# Autodesk Inventor assembly: Assembly1
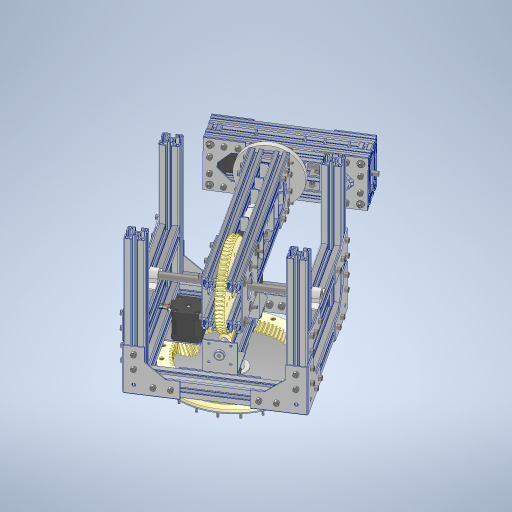
[picture p0: Inventor's stored thumbnail of the model, 512x512]
Saved by Autodesk Inventor 2024 (Build 280153000, 153)
## iProperties
Created: 2025-12-08
Part Number: Assembly1
Document SubType Name: Assembly
Designer: schar
Author: schar
## Documents named in this file (47)
- C:\Users\schar\Desktop\projectBlueprint\AMSTS\hardware\Assembly1.iam
- C:\Users\schar\Desktop\projectBlueprint\AMSTS\hardware\3030_200.ipt
- C:\Users\schar\Desktop\projectBlueprint\AMSTS\hardware\Connect2x3030_m6.ipt
- C:\Users\schar\Desktop\projectBlueprint\AMSTS\hardware\3030_tnut_m6.ipt
- C:\Users\schar\Documents\Inventor\Content Center Files\R2024\en-US\AS 1420\AS 1420 - 1973 - M5 x 10.ipt
- C:\Users\schar\Desktop\projectBlueprint\AMSTS\hardware\3030_260.ipt
- C:\Users\schar\Desktop\projectBlueprint\AMSTS\hardware\3030_connector_assembled.iam
- C:\Users\schar\Desktop\projectBlueprint\AMSTS\hardware\3030_connector_assembled_MIR.iam
- C:\Users\schar\Desktop\projectBlueprint\AMSTS\hardware\3030_connector_assembled_MIR1.iam
- C:\Users\schar\Desktop\projectBlueprint\AMSTS\hardware\3030_connector_assembled_MIR_MIR.iam
- C:\Users\schar\Desktop\projectBlueprint\AMSTS\hardware\3030_T_connector_assembled.iam
- C:\Users\schar\Desktop\projectBlueprint\AMSTS\hardware\3030_T_connector_assembled_MIR1.iam
- C:\Users\schar\Desktop\projectBlueprint\AMSTS\hardware\wormgear_pol_base.iam
- C:\Users\schar\Desktop\projectBlueprint\AMSTS\hardware\base_axis_static_12mm.ipt
- C:\Users\schar\Desktop\projectBlueprint\AMSTS\hardware\base_axis_12mm.ipt
- C:\Users\schar\Desktop\projectBlueprint\AMSTS\hardware\NEMA17-3030-m6-holder.ipt
- C:\Users\schar\Desktop\projectBlueprint\AMSTS\hardware\3030_tnut_m6_main.ipt
- C:\Users\schar\Desktop\projectBlueprint\AMSTS\hardware\basis-bearing-3030-m6-holder.ipt
- C:\Users\schar\Desktop\projectBlueprint\AMSTS\hardware\wormgear_axis_6mm.ipt
- C:\Users\schar\Desktop\projectBlueprint\AMSTS\hardware\wormgear_worm_axes_holder.ipt
- C:\Users\schar\Desktop\projectBlueprint\AMSTS\hardware\bearing_shaft_base_mount.ipt
- C:\Users\schar\Desktop\projectBlueprint\AMSTS\hardware\az_rot_plate.iam
- C:\Users\schar\Desktop\projectBlueprint\AMSTS\hardware\the_part_that_holds_everything_together.ipt
- C:\Users\schar\Desktop\projectBlueprint\AMSTS\hardware\6901.iam
- C:\Users\schar\Desktop\projectBlueprint\AMSTS\hardware\2020_400.ipt
- C:\Users\schar\Desktop\projectBlueprint\AMSTS\hardware\mount_plate_4x2020.ipt
- C:\Users\schar\Documents\Inventor\Content Center Files\R2024\en-US\DIN 9021\DIN 9021 - 5,3.ipt
- C:\Users\schar\Desktop\projectBlueprint\AMSTS\hardware\m5x70.ipt
- C:\Users\schar\Desktop\projectBlueprint\AMSTS\hardware\3030_tnut_m6_MIR3.ipt
- C:\Users\schar\Documents\Inventor\Content Center Files\R2024\en-US\ISO 4762(1)\DIN EN ISO 4762 - M6 x 10.ipt
- C:\Users\schar\Desktop\projectBlueprint\AMSTS\hardware\3030_L-Bracket_asm.ipt.iam
- C:\Users\schar\Desktop\projectBlueprint\AMSTS\hardware\4x2020_in.iam
- C:\Users\schar\Desktop\projectBlueprint\AMSTS\hardware\2020_4x2020_hz.ipt
- C:\Users\schar\Desktop\projectBlueprint\AMSTS\hardware\2020_4x2020_ve.ipt
- C:\Users\schar\Desktop\projectBlueprint\AMSTS\hardware\17HE19-2004S.ipt
- C:\Users\schar\Desktop\projectBlueprint\AMSTS\hardware\az_rot_mot_asm.ipt.iam
- C:\Users\schar\Desktop\projectBlueprint\AMSTS\hardware\azimuth_gear_in.ipt
- C:\Users\schar\Documents\Inventor\Content Center Files\R2024\en-US\DIN 913\DIN 913 - M5 x 5.ipt
- C:\Users\schar\Desktop\projectBlueprint\AMSTS\hardware\Connect_u2020_asm.iam
- C:\Users\schar\Desktop\projectBlueprint\AMSTS\hardware\m4x70_example.ipt
- C:\Users\schar\Documents\Inventor\Content Center Files\R2024\en-US\DIN 9021\DIN 9021 - 4,3.ipt
- C:\Users\schar\Desktop\projectBlueprint\AMSTS\hardware\ax4_holder_asm.iam
- C:\Users\schar\Desktop\projectBlueprint\AMSTS\hardware\4ax_plate_joint_asm.iam
- C:\Users\schar\Desktop\projectBlueprint\AMSTS\hardware\ax4.iam
- C:\Users\schar\Desktop\projectBlueprint\AMSTS\hardware\13to6_bearing.ipt
- 3030_L-Bracket_asm.ipt
- az_rot_mot_asm.ipt
## Components (125 placed, 44 different names)
1. 3030_tnut_m6_main:17 — Rotational:21
2. 3030_tnut_m6_main:18 — Rotational:22
3. bearing_shaft_base_mount:1 — Mate:102, Flush:37, Flush:38, Rotational:21, Rotational:22, Mate:103, Rotational:25
4. az_rot_plate:1 [sub-assembly] — Mate:103, Tangent:1, Rotational:23, Rotational:24, Mate:182, Insert:27, Mate:183
5. the_part_that_holds_everything_together:1 — Rotational:24, Rotational:25
6. 6901:1 [sub-assembly] — Rotational:23
7. 2020_400:1 — Mate:109, Mate:113, Mate:114, Mate:121, Mate:157, Mate:158, Mate:162, Flush:46, Flush:47, Mate:185, Mate:187, Flush:63
8. 2020_400:2 — Mate:107, Mate:117, Mate:118, Mate:122, Mate:123, Flush:56, Mate:184
9. 2020_400:3 — Mate:110, Mate:111, Mate:112, Mate:124, Flush:43, Mate:155, Mate:161, Flush:44, Flush:45
10. 2020_400:4 — Mate:108, Mate:115, Mate:116, Mate:119, Mate:120, Mate:159, Mate:160, Flush:58, Mate:186, Flush:62
11. mount_plate_4x2020:1 — Mate:119, Mate:120, Mate:121, Mate:125, Mate:150
12. mount_plate_4x2020:2 — Mate:122, Mate:123, Mate:124, Mate:154
13. 3030_L-Bracket_asm.ipt:1 [sub-assembly] — Mate:141, Flush:41, Mate:142
14. 3030_L-Bracket_asm.ipt:2 [sub-assembly] — Mate:139, Flush:40, Mate:140
15. 3030_L-Bracket_asm.ipt:3 [sub-assembly] — Mate:137, Flush:39, Mate:138
16. 3030_L-Bracket_asm.ipt:4 [sub-assembly] — Mate:143, Flush:42, Mate:144
17. 4x2020_in:1 [sub-assembly] — Flush:43, Mate:155, Mate:156, Mate:194, Mate:195, Mate:197
18. 2020_4x2020_hz:1 — Mate:159, Mate:160, Flush:62
19. 2020_4x2020_hz:2 — Mate:157, Mate:158, Flush:63
20. 2020_4x2020_ve:1 — Mate:162, Flush:46, Flush:47, Flush:59
21. 2020_4x2020_ve:2 — Mate:161, Flush:44, Flush:45, Flush:57, Mate:196
22. 17HE19-2004S:1 — Mate:165, Mate:166, Mate:167, Mate:202
23. az_rot_mot_asm.ipt:1 [sub-assembly] — Mate:181, Flush:55, Mate:182
24. 3030_tnut_m6_MIR3:1 — Mate:177, Mate:178
25. 3030_tnut_m6_MIR3:2 — Mate:179, Mate:180
26. DIN EN ISO 4762 M6 x 10:1 — Mate:174, Mate:175, Mate:177
27. DIN EN ISO 4762 M6 x 10:2 — Mate:173, Mate:176, Mate:179
28. azimuth_gear_in:1 — Rotational:31, Insert:27, Mate:183
29. DIN 913 M5 x 5:1 — Rotational:31
30. Connect_u2020_asm:1 [sub-assembly] — Flush:56, Flush:57, Mate:184, Mate:192, Mate:193
31. Connect_u2020_asm:2 [sub-assembly] — Flush:58, Flush:59, Mate:185, Mate:188, Mate:189
32. m4x70_example:1 — Mate:187, Mate:188, Mate:191
33. m4x70_example:2 — Mate:186, Mate:189, Mate:190
34. DIN 9021 4,3:1 — Mate:190, Mate:193
35. DIN 9021 4,3:2 — Mate:191, Mate:192
36. ax4_holder_asm:1 [sub-assembly] — Mate:194, Mate:195, Flush:60, Mate:198, Mate:205
37. 4ax_plate_joint_asm:1 [sub-assembly] — Mate:196, Mate:197
38. ax4:1 [sub-assembly] — Flush:60, Mate:198, Mate:205
39. 13to6_bearing:1 — Mate:200, Flush:64, Flush:65
40. 3030_200:1 — Mate:1, Mate:2, Flush:1, Flush:2, Mate:4, Flush:5, Flush:6, Mate:30, Mate:48, Mate:141, Flush:41, Mate:143, Flush:42, Flush:52, Mate:203
41. 3030_200:2 — Mate:3, Flush:3, Flush:4, Mate:6, Flush:9, Flush:10
42. Connect2x3030_m6:1 — Mate:1, Mate:2, Flush:1, Flush:2, Mate:3, Flush:3, Flush:4, Rigid:1, Rotational:5, Rotational:6, Rotational:7, Insert:11, Insert:12, Insert:14, Insert:15, Mate:19, Mate:20, Mate:21, Mate:36, Mate:37
43. Connect2x3030_m6:2 — Mate:4, Flush:5, Flush:6, Mate:5, Flush:7, Flush:8, Rotational:1, Rotational:2, Rotational:3, Rotational:4, Insert:6, Insert:7, Insert:9, Insert:10, Mate:10, Mate:11, Mate:12, Mate:32, Mate:33
44. Connect2x3030_m6:3 — Mate:8, Flush:11, Flush:12, Rotational:12, Rotational:13, Rotational:14, Rotational:15, Insert:1, Insert:2, Insert:4, Insert:5, Mate:13, Mate:14, Mate:15, Mate:40, Mate:41
45. Connect2x3030_m6:4 — Mate:6, Flush:9, Flush:10, Mate:7, Flush:13, Mate:9, Flush:14, Rotational:8, Rotational:9, Rotational:10, Rotational:11, Insert:16, Insert:17, Insert:18, Insert:20, Mate:16, Mate:17, Mate:18, Mate:23, Flush:15, Mate:25
46. 3030_200:3 — Mate:5, Flush:7, Flush:8, Mate:8, Flush:11, Flush:12, Mate:52, Angle:1, Mate:181, Flush:55
47. 3030_200:4 — Flush:13, Mate:9, Flush:14, Mate:53, Flush:23, Mate:137, Flush:39, Mate:139, Flush:40
48. 3030_connector_assembled:1 [sub-assembly] — Mate:24, Mate:25, Mate:26
49. 3030_connector_assembled:2 [sub-assembly] — Mate:22, Mate:23, Flush:15, Mate:26
50. 3030_connector_assembled_MIR:1 [sub-assembly] — Mate:27, Mate:39, Mate:40
51. 3030_connector_assembled_MIR:2 [sub-assembly] — Mate:27, Mate:38, Mate:41
52. 3030_connector_assembled_MIR1:1 [sub-assembly] — Mate:28, Mate:34, Mate:37
53. 3030_connector_assembled_MIR1:2 [sub-assembly] — Mate:28, Mate:35, Mate:36
54. 3030_connector_assembled_MIR_MIR:1 [sub-assembly] — Mate:29, Mate:30, Mate:33
55. 3030_connector_assembled_MIR_MIR:2 [sub-assembly] — Mate:29, Mate:31, Mate:32, Mate:170
56. 3030_260:1 — Mate:10, Mate:11, Mate:12, Mate:31, Mate:49, Flush:20
57. 3030_260:2 — Mate:13, Mate:14, Mate:15, Mate:38, Mate:39, Mate:42, Flush:16
58. 3030_260:3 — Mate:16, Mate:17, Mate:18, Mate:22, Mate:24, Mate:43, Flush:17, Mate:204
59. 3030_260:4 — Mate:19, Mate:20, Mate:21, Mate:34, Mate:35, Mate:50, Flush:21
60. wormgear_axis_6mm:1 — Mate:63, Mate:64, Mate:65, Flush:65, Mate:202
61. wormgear_worm_axes_holder:1 — Mate:64, Mate:65, Rotational:26
62. wormgear_pol_base:1 [sub-assembly] — Rigid:2, Mate:63, Rotational:26, Mate:107, Mate:108, Mate:109, Mate:110, Mate:111, Mate:112, Mate:113, Mate:114, Mate:115, Mate:116, Mate:117, Mate:118, Mate:156
63. base_axis_static_12mm:1 — Flush:30, Mate:57, Insert:22
64. base_axis_static_12mm:2 — Mate:58, Flush:31, Insert:21, Mate:201
65. base_axis_12mm:1 — Insert:21, Insert:22, Rigid:2
66. basis-bearing-3030-m6-holder:1 — Mate:172, Flush:54, Mate:173, Mate:174, Mate:175, Mate:176, Mate:200, Flush:64, Mate:203
67. NEMA17-3030-m6-holder:1 — Mate:59, Flush:33, Mate:165, Mate:166, Mate:167
68. 3030_T_connector_assembled:1 [sub-assembly] — Mate:43, Flush:17, Mate:56, Flush:29
69. 3030_T_connector_assembled:2 [sub-assembly] — Mate:42, Flush:16, Flush:26
70. 3030_T_connector_assembled_MIR1:1 [sub-assembly] — Mate:50, Flush:21, Mate:55, Flush:27, Flush:28
71. 3030_T_connector_assembled_MIR1:2 [sub-assembly] — Mate:49, Flush:20, Mate:54, Flush:24, Flush:25, Mate:170
72. 3030_200:5 — Mate:48, Mate:52, Flush:22, Mate:59, Flush:33, Mate:102, Flush:37, Flush:38, Mate:138, Mate:140, Mate:142, Mate:144, Flush:52, Mate:172, Flush:54, Mate:178, Mate:180
73. 3030_T_connector_assembled:4 [sub-assembly] — Mate:53, Flush:22, Flush:23
74. 3030_200:6 — Mate:55, Flush:27, Flush:28, Mate:56, Flush:29, Flush:30, Mate:57
75. 3030_200:7 — Mate:54, Flush:24, Flush:25, Flush:26, Mate:58, Flush:31, Mate:201
76. 3030_tnut_m6:1 — Rotational:12
77. 3030_tnut_m6:2 — Rotational:11
78. 3030_tnut_m6:3 — Rigid:1
79. 3030_tnut_m6:4 — Rotational:1
80. 3030_tnut_m6:5 — Rotational:13
81. 3030_tnut_m6:6 — Rotational:10
82. 3030_tnut_m6:7 — Rotational:5
83. 3030_tnut_m6:8 — Rotational:2
84. 3030_tnut_m6:9 — Rotational:15
85. 3030_tnut_m6:10 — Rotational:8
86. 3030_tnut_m6:11 — Rotational:6
87. 3030_tnut_m6:12 — Rotational:4
88. 3030_tnut_m6:13 — Rotational:14
89. 3030_tnut_m6:14 — Rotational:9
90. 3030_tnut_m6:15 — Rotational:7
91. 3030_tnut_m6:16 — Rotational:3
92. AS 1420 - Metric M5 x 10:1 — Insert:1
93. AS 1420 - Metric M5 x 10:2 — Insert:2
94. AS 1420 - Metric M5 x 10:4 — Insert:4
95. AS 1420 - Metric M5 x 10:5 — Insert:5
96. AS 1420 - Metric M5 x 10:6 — Insert:6
97. AS 1420 - Metric M5 x 10:7 — Insert:7
98. AS 1420 - Metric M5 x 10:9 — Insert:9
99. AS 1420 - Metric M5 x 10:10 — Insert:10
100. AS 1420 - Metric M5 x 10:11 — Insert:11
101. AS 1420 - Metric M5 x 10:12 — Insert:12
102. AS 1420 - Metric M5 x 10:14 — Insert:14
103. AS 1420 - Metric M5 x 10:15 — Insert:15
104. AS 1420 - Metric M5 x 10:16 — Insert:16
105. AS 1420 - Metric M5 x 10:17 — Insert:17
106. AS 1420 - Metric M5 x 10:18 — Insert:18
107. AS 1420 - Metric M5 x 10:20 — Insert:20
108. m5x70:1 — Mate:125, Mate:150
109. m5x70:2
110. m5x70:3
111. m5x70:4
112. m5x70:5 — Mate:151, Mate:152, Mate:153
113. m5x70:6
114. DIN 9021 5,3:1 — Mate:151, Mate:152
115. DIN 9021 5,3:2
116. DIN 9021 5,3:3
117. DIN 9021 5,3:4
118. DIN 9021 5,3:5
119. DIN 9021 5,3:6
120. DIN 9021 5,3:7 — Mate:153, Mate:154
121. DIN 9021 5,3:8
122. DIN 9021 5,3:9
123. DIN 9021 5,3:10
124. DIN 9021 5,3:11
125. DIN 9021 5,3:12
## Component patterns: (6 elements, first: m5x70:1), (6 elements, first: DIN 9021 5,3:1), (6 elements, first: DIN 9021 5,3:7)
## Relationships (234: Mate 136, Flush 53, RevoluteJoint 22, Insert 19, WeldJoint 2, Angle 1, Tangent 1)
- Mate:1: 3030_200:1 ↔ Connect2x3030_m6:1
- Mate:2: 3030_200:1 ↔ Connect2x3030_m6:1
- Flush:1: 3030_200:1 ↔ Connect2x3030_m6:1
- Flush:2 (30 mm): 3030_200:1 ↔ Connect2x3030_m6:1
- Mate:3: 3030_200:2 ↔ Connect2x3030_m6:1
- Flush:3 (30 mm): 3030_200:2 ↔ Connect2x3030_m6:1
- Flush:4: 3030_200:2 ↔ Connect2x3030_m6:1
- Mate:4: 3030_200:1 ↔ Connect2x3030_m6:2
- Flush:5 (-30 mm): 3030_200:1 ↔ Connect2x3030_m6:2
- Flush:6: 3030_200:1 ↔ Connect2x3030_m6:2
- Mate:5: Connect2x3030_m6:2 ↔ 3030_200:3
- Flush:7 (30 mm): Connect2x3030_m6:2 ↔ 3030_200:3
- Flush:8: Connect2x3030_m6:2 ↔ 3030_200:3
- Mate:6: 3030_200:2 ↔ Connect2x3030_m6:4
- Flush:9 (-30 mm): 3030_200:2 ↔ Connect2x3030_m6:4
- Flush:10: 3030_200:2 ↔ Connect2x3030_m6:4
- Mate:7: Connect2x3030_m6:4
- Mate:8: Connect2x3030_m6:3 ↔ 3030_200:3
- Flush:11 (-30 mm): Connect2x3030_m6:3 ↔ 3030_200:3
- Flush:12: Connect2x3030_m6:3 ↔ 3030_200:3
- Flush:13: Connect2x3030_m6:4 ↔ 3030_200:4
- Mate:9: Connect2x3030_m6:4 ↔ 3030_200:4
- Flush:14 (-30 mm): Connect2x3030_m6:4 ↔ 3030_200:4
- Rotational:1 [RevoluteJoint] (-0.357 mm): Connect2x3030_m6:2 ↔ 3030_tnut_m6:4
- Rotational:2 [RevoluteJoint] (-0.357 mm): Connect2x3030_m6:2 ↔ 3030_tnut_m6:8
- Rotational:3 [RevoluteJoint] (-0.357 mm): Connect2x3030_m6:2 ↔ 3030_tnut_m6:16
- Rotational:4 [RevoluteJoint] (-0.357 mm): Connect2x3030_m6:2 ↔ 3030_tnut_m6:12
- Rigid:1 [WeldJoint] (-0.357 mm): Connect2x3030_m6:1 ↔ 3030_tnut_m6:3
- Rotational:5 [RevoluteJoint] (-0.357 mm): Connect2x3030_m6:1 ↔ 3030_tnut_m6:7
- Rotational:6 [RevoluteJoint] (-0.357 mm): Connect2x3030_m6:1 ↔ 3030_tnut_m6:11
- Rotational:7 [RevoluteJoint] (-0.357 mm): Connect2x3030_m6:1 ↔ 3030_tnut_m6:15
- Rotational:8 [RevoluteJoint] (-0.357 mm): Connect2x3030_m6:4 ↔ 3030_tnut_m6:10
- Rotational:9 [RevoluteJoint] (-0.357 mm): Connect2x3030_m6:4 ↔ 3030_tnut_m6:14
- Rotational:10 [RevoluteJoint] (-0.357 mm): Connect2x3030_m6:4 ↔ 3030_tnut_m6:6
- Rotational:11 [RevoluteJoint] (-0.357 mm): Connect2x3030_m6:4 ↔ 3030_tnut_m6:2
- Rotational:12 [RevoluteJoint] (-0.357 mm): Connect2x3030_m6:3 ↔ 3030_tnut_m6:1
- Rotational:13 [RevoluteJoint]: Connect2x3030_m6:3 ↔ 3030_tnut_m6:5
- Rotational:14 [RevoluteJoint] (-0.357 mm): Connect2x3030_m6:3 ↔ 3030_tnut_m6:13
- Rotational:15 [RevoluteJoint] (-0.357 mm): Connect2x3030_m6:3 ↔ 3030_tnut_m6:9
- Insert:1: Connect2x3030_m6:3 ↔ AS 1420 - Metric M5 x 10:1
- Insert:2: Connect2x3030_m6:3 ↔ AS 1420 - Metric M5 x 10:2
- Insert:4: Connect2x3030_m6:3 ↔ AS 1420 - Metric M5 x 10:4
- Insert:5: Connect2x3030_m6:3 ↔ AS 1420 - Metric M5 x 10:5
- Insert:6: Connect2x3030_m6:2 ↔ AS 1420 - Metric M5 x 10:6
- Insert:7: Connect2x3030_m6:2 ↔ AS 1420 - Metric M5 x 10:7
- Insert:9: Connect2x3030_m6:2 ↔ AS 1420 - Metric M5 x 10:9
- Insert:10: Connect2x3030_m6:2 ↔ AS 1420 - Metric M5 x 10:10
- Insert:11: Connect2x3030_m6:1 ↔ AS 1420 - Metric M5 x 10:11
- Insert:12: Connect2x3030_m6:1 ↔ AS 1420 - Metric M5 x 10:12
- Insert:14: Connect2x3030_m6:1 ↔ AS 1420 - Metric M5 x 10:14
- Insert:15: Connect2x3030_m6:1 ↔ AS 1420 - Metric M5 x 10:15
- Insert:16: Connect2x3030_m6:4 ↔ AS 1420 - Metric M5 x 10:16
- Insert:17: Connect2x3030_m6:4 ↔ AS 1420 - Metric M5 x 10:17
- Insert:18: Connect2x3030_m6:4 ↔ AS 1420 - Metric M5 x 10:18
- Insert:20: Connect2x3030_m6:4 ↔ AS 1420 - Metric M5 x 10:20
- Mate:10: Connect2x3030_m6:2 ↔ 3030_260:1
- Mate:11: Connect2x3030_m6:2 ↔ 3030_260:1
- Mate:12: Connect2x3030_m6:2 ↔ 3030_260:1
- Mate:13: Connect2x3030_m6:3 ↔ 3030_260:2
- Mate:14: Connect2x3030_m6:3 ↔ 3030_260:2
- Mate:15: Connect2x3030_m6:3 ↔ 3030_260:2
- Mate:16: Connect2x3030_m6:4 ↔ 3030_260:3
- Mate:17: Connect2x3030_m6:4 ↔ 3030_260:3
- Mate:18: Connect2x3030_m6:4 ↔ 3030_260:3
- Mate:19: Connect2x3030_m6:1 ↔ 3030_260:4
- Mate:20: Connect2x3030_m6:1 ↔ 3030_260:4
- Mate:21: Connect2x3030_m6:1 ↔ 3030_260:4
- Mate:22: 3030_connector_assembled:2 ↔ 3030_260:3
- Mate:23: Connect2x3030_m6:4 ↔ 3030_connector_assembled:2
- Flush:15: Connect2x3030_m6:4 ↔ 3030_connector_assembled:2
- Mate:24: 3030_connector_assembled:1 ↔ 3030_260:3
- Mate:25: Connect2x3030_m6:4 ↔ 3030_connector_assembled:1
- Mate:26: 3030_connector_assembled:1 ↔ 3030_connector_assembled:2
- Mate:27: 3030_connector_assembled_MIR:1 ↔ 3030_connector_assembled_MIR:2
- Mate:28: 3030_connector_assembled_MIR1:1 ↔ 3030_connector_assembled_MIR1:2
- Mate:29: 3030_connector_assembled_MIR_MIR:1 ↔ 3030_connector_assembled_MIR_MIR:2
- Mate:30: 3030_200:1 ↔ 3030_connector_assembled_MIR_MIR:1
- Mate:31: 3030_connector_assembled_MIR_MIR:2 ↔ 3030_260:1
- Mate:32: Connect2x3030_m6:2 ↔ 3030_connector_assembled_MIR_MIR:2
- Mate:33: Connect2x3030_m6:2 ↔ 3030_connector_assembled_MIR_MIR:1
- Mate:34: 3030_connector_assembled_MIR1:1 ↔ 3030_260:4
- Mate:35: 3030_connector_assembled_MIR1:2 ↔ 3030_260:4
- Mate:36: Connect2x3030_m6:1 ↔ 3030_connector_assembled_MIR1:2
- Mate:37: Connect2x3030_m6:1 ↔ 3030_connector_assembled_MIR1:1
- Mate:38: 3030_connector_assembled_MIR:2 ↔ 3030_260:2
- Mate:39: 3030_connector_assembled_MIR:1 ↔ 3030_260:2
- Mate:40: Connect2x3030_m6:3 ↔ 3030_connector_assembled_MIR:1
- Mate:41: Connect2x3030_m6:3 ↔ 3030_connector_assembled_MIR:2
- Mate:42: 3030_260:2 ↔ 3030_T_connector_assembled:2
- Flush:16: 3030_260:2 ↔ 3030_T_connector_assembled:2
- Mate:43: 3030_260:3 ↔ 3030_T_connector_assembled:1
- Flush:17: 3030_260:3 ↔ 3030_T_connector_assembled:1
- Mate:48: 3030_200:1 ↔ 3030_200:5
- Mate:49: 3030_260:1 ↔ 3030_T_connector_assembled_MIR1:2
- Flush:20: 3030_260:1 ↔ 3030_T_connector_assembled_MIR1:2
- Mate:50: 3030_260:4 ↔ 3030_T_connector_assembled_MIR1:1
- Flush:21: 3030_260:4 ↔ 3030_T_connector_assembled_MIR1:1
- Mate:52 (85 mm): 3030_200:3 ↔ 3030_200:5
- Mate:53: 3030_200:4 ↔ 3030_T_connector_assembled:4
- Flush:22: 3030_200:5 ↔ 3030_T_connector_assembled:4
- Flush:23: 3030_200:4 ↔ 3030_T_connector_assembled:4
- Mate:54: 3030_T_connector_assembled_MIR1:2 ↔ 3030_200:7
- Flush:24: 3030_T_connector_assembled_MIR1:2 ↔ 3030_200:7
- Flush:25 (-30 mm): 3030_T_connector_assembled_MIR1:2 ↔ 3030_200:7
- Flush:26: 3030_T_connector_assembled:2 ↔ 3030_200:7
- Mate:55: 3030_T_connector_assembled_MIR1:1 ↔ 3030_200:6
- Flush:27: 3030_T_connector_assembled_MIR1:1 ↔ 3030_200:6
- Flush:28 (30 mm): 3030_T_connector_assembled_MIR1:1 ↔ 3030_200:6
- Mate:56: 3030_T_connector_assembled:1 ↔ 3030_200:6
- Flush:29: 3030_T_connector_assembled:1 ↔ 3030_200:6
- Flush:30: base_axis_static_12mm:1 ↔ 3030_200:6
- Mate:57: base_axis_static_12mm:1 ↔ 3030_200:6
- Mate:58: base_axis_static_12mm:2 ↔ 3030_200:7
- Flush:31: base_axis_static_12mm:2 ↔ 3030_200:7
- Insert:21: base_axis_static_12mm:2 ↔ base_axis_12mm:1
- Insert:22: base_axis_static_12mm:1 ↔ base_axis_12mm:1
- Rigid:2 [WeldJoint] (5 mm): wormgear_pol_base:1 ↔ base_axis_12mm:1
- Mate:59: NEMA17-3030-m6-holder:1 ↔ 3030_200:5
- Flush:33 (-10 mm): NEMA17-3030-m6-holder:1 ↔ 3030_200:5
- Mate:63: wormgear_axis_6mm:1 ↔ wormgear_pol_base:1
- Mate:64: wormgear_axis_6mm:1 ↔ wormgear_worm_axes_holder:1
- Mate:65: wormgear_axis_6mm:1 ↔ wormgear_worm_axes_holder:1
- Mate:102: bearing_shaft_base_mount:1 ↔ 3030_200:5
- Flush:37 (79 mm): bearing_shaft_base_mount:1 ↔ 3030_200:5
- Flush:38: bearing_shaft_base_mount:1 ↔ 3030_200:5
- Rotational:21 [RevoluteJoint] (0.357 mm): 3030_tnut_m6_main:17 ↔ bearing_shaft_base_mount:1
- Rotational:22 [RevoluteJoint] (0.357 mm): 3030_tnut_m6_main:18 ↔ bearing_shaft_base_mount:1
- Mate:103: bearing_shaft_base_mount:1 ↔ az_rot_plate:1
- Angle:1 (0 deg): 3030_200:3
- Tangent:1: az_rot_plate:1
- Rotational:23 [RevoluteJoint]: az_rot_plate:1 ↔ 6901:1
- Rotational:24 [RevoluteJoint]: az_rot_plate:1 ↔ the_part_that_holds_everything_together:1
- Rotational:25 [RevoluteJoint]: bearing_shaft_base_mount:1 ↔ the_part_that_holds_everything_together:1
- Rotational:26 [RevoluteJoint]: wormgear_worm_axes_holder:1 ↔ wormgear_pol_base:1
- Mate:107: 2020_400:2 ↔ wormgear_pol_base:1
- Mate:108: 2020_400:4 ↔ wormgear_pol_base:1
- Mate:109: 2020_400:1 ↔ wormgear_pol_base:1
- Mate:110: 2020_400:3 ↔ wormgear_pol_base:1
- Mate:111: 2020_400:3 ↔ wormgear_pol_base:1
- Mate:112: 2020_400:3 ↔ wormgear_pol_base:1
- Mate:113: 2020_400:1 ↔ wormgear_pol_base:1
- Mate:114: 2020_400:1 ↔ wormgear_pol_base:1
- Mate:115: 2020_400:4 ↔ wormgear_pol_base:1
- Mate:116: 2020_400:4 ↔ wormgear_pol_base:1
- Mate:117: 2020_400:2 ↔ wormgear_pol_base:1
- Mate:118: 2020_400:2 ↔ wormgear_pol_base:1
- Mate:119: 2020_400:4 ↔ mount_plate_4x2020:1
- Mate:120: 2020_400:4 ↔ mount_plate_4x2020:1
- Mate:121: 2020_400:1 ↔ mount_plate_4x2020:1
- Mate:122: 2020_400:2 ↔ mount_plate_4x2020:2
- Mate:123: 2020_400:2 ↔ mount_plate_4x2020:2
- Mate:124: 2020_400:3 ↔ mount_plate_4x2020:2
- Mate:125: mount_plate_4x2020:1 ↔ m5x70:1
- Mate:137: 3030_L-Bracket_asm.ipt:3 ↔ 3030_200:4
- Flush:39: 3030_L-Bracket_asm.ipt:3 ↔ 3030_200:4
- Mate:138: 3030_L-Bracket_asm.ipt:3 ↔ 3030_200:5
- Mate:139: 3030_L-Bracket_asm.ipt:2 ↔ 3030_200:4
- Flush:40: 3030_L-Bracket_asm.ipt:2 ↔ 3030_200:4
- Mate:140: 3030_L-Bracket_asm.ipt:2 ↔ 3030_200:5
- Mate:141: 3030_L-Bracket_asm.ipt:1 ↔ 3030_200:1
- Flush:41: 3030_L-Bracket_asm.ipt:1 ↔ 3030_200:1
- Mate:142: 3030_L-Bracket_asm.ipt:1 ↔ 3030_200:5
- Mate:143: 3030_L-Bracket_asm.ipt:4 ↔ 3030_200:1
- Flush:42: 3030_L-Bracket_asm.ipt:4 ↔ 3030_200:1
- Mate:144: 3030_L-Bracket_asm.ipt:4 ↔ 3030_200:5
- Mate:150 (1.2 mm): mount_plate_4x2020:1 ↔ m5x70:1
- Mate:151: m5x70:5 ↔ DIN 9021 5,3:1
- Mate:152: m5x70:5 ↔ DIN 9021 5,3:1
- Mate:153: m5x70:5 ↔ DIN 9021 5,3:7
- Mate:154: mount_plate_4x2020:2 ↔ DIN 9021 5,3:7
- Flush:43: 2020_400:3 ↔ 4x2020_in:1
- Mate:155: 2020_400:3 ↔ 4x2020_in:1
- Mate:156 (50.56 mm): 4x2020_in:1 ↔ wormgear_pol_base:1
- Mate:157: 2020_400:1 ↔ 2020_4x2020_hz:2
- Mate:158: 2020_400:1 ↔ 2020_4x2020_hz:2
- Mate:159: 2020_400:4 ↔ 2020_4x2020_hz:1
- Mate:160: 2020_400:4 ↔ 2020_4x2020_hz:1
- Mate:161: 2020_400:3 ↔ 2020_4x2020_ve:2
- Flush:44: 2020_400:3 ↔ 2020_4x2020_ve:2
- Flush:45: 2020_400:3 ↔ 2020_4x2020_ve:2
- Mate:162: 2020_400:1 ↔ 2020_4x2020_ve:1
- Flush:46: 2020_400:1 ↔ 2020_4x2020_ve:1
- Flush:47: 2020_400:1 ↔ 2020_4x2020_ve:1
- Mate:165: 17HE19-2004S:1 ↔ NEMA17-3030-m6-holder:1
- Mate:166: 17HE19-2004S:1 ↔ NEMA17-3030-m6-holder:1
- Mate:167: 17HE19-2004S:1 ↔ NEMA17-3030-m6-holder:1
- Flush:52: 3030_200:1 ↔ 3030_200:5
- Mate:170 (6.262 mm): 3030_connector_assembled_MIR_MIR:2 ↔ 3030_T_connector_assembled_MIR1:2
- Mate:172: basis-bearing-3030-m6-holder:1 ↔ 3030_200:5
- Flush:54 (-10 mm): basis-bearing-3030-m6-holder:1 ↔ 3030_200:5
- Mate:173: DIN EN ISO 4762 M6 x 10:2 ↔ basis-bearing-3030-m6-holder:1
- Mate:174: DIN EN ISO 4762 M6 x 10:1 ↔ basis-bearing-3030-m6-holder:1
- Mate:175: DIN EN ISO 4762 M6 x 10:1 ↔ basis-bearing-3030-m6-holder:1
- Mate:176: DIN EN ISO 4762 M6 x 10:2 ↔ basis-bearing-3030-m6-holder:1
- Mate:177: 3030_tnut_m6_MIR3:1 ↔ DIN EN ISO 4762 M6 x 10:1
- Mate:178: 3030_tnut_m6_MIR3:1 ↔ 3030_200:5
- Mate:179: 3030_tnut_m6_MIR3:2 ↔ DIN EN ISO 4762 M6 x 10:2
- Mate:180: 3030_tnut_m6_MIR3:2 ↔ 3030_200:5
- Mate:181: az_rot_mot_asm.ipt:1 ↔ 3030_200:3
- Flush:55: az_rot_mot_asm.ipt:1 ↔ 3030_200:3
- Mate:182: az_rot_plate:1 ↔ az_rot_mot_asm.ipt:1
- Rotational:31 [RevoluteJoint]: azimuth_gear_in:1 ↔ DIN 913 M5 x 5:1
- Insert:27: az_rot_plate:1 ↔ azimuth_gear_in:1
- Mate:183: az_rot_plate:1 ↔ azimuth_gear_in:1
- Flush:56: 2020_400:2 ↔ Connect_u2020_asm:1
- Flush:57: 2020_4x2020_ve:2 ↔ Connect_u2020_asm:1
- Mate:184: 2020_400:2 ↔ Connect_u2020_asm:1
- Flush:58: 2020_400:4 ↔ Connect_u2020_asm:2
- Flush:59: 2020_4x2020_ve:1 ↔ Connect_u2020_asm:2
- Mate:185: 2020_400:1 ↔ Connect_u2020_asm:2
- Mate:186: 2020_400:4 ↔ m4x70_example:2
- Mate:187: 2020_400:1 ↔ m4x70_example:1
- Mate:188: Connect_u2020_asm:2 ↔ m4x70_example:1
- Mate:189: Connect_u2020_asm:2 ↔ m4x70_example:2
- Mate:190: m4x70_example:2 ↔ DIN 9021 4,3:1
- Mate:191: m4x70_example:1 ↔ DIN 9021 4,3:2
- Mate:192: Connect_u2020_asm:1 ↔ DIN 9021 4,3:2
- Mate:193: Connect_u2020_asm:1 ↔ DIN 9021 4,3:1
- Mate:194: 4x2020_in:1 ↔ ax4_holder_asm:1
- Mate:195: 4x2020_in:1 ↔ ax4_holder_asm:1
- Mate:196: 2020_4x2020_ve:2 ↔ 4ax_plate_joint_asm:1
- Mate:197: 4x2020_in:1 ↔ 4ax_plate_joint_asm:1
- Flush:60: ax4_holder_asm:1 ↔ ax4:1
- Mate:198: ax4_holder_asm:1 ↔ ax4:1
- Flush:62: 2020_400:4 ↔ 2020_4x2020_hz:1
- Flush:63: 2020_400:1 ↔ 2020_4x2020_hz:2
- Mate:200: 13to6_bearing:1 ↔ basis-bearing-3030-m6-holder:1
- Flush:64: 13to6_bearing:1 ↔ basis-bearing-3030-m6-holder:1
- Mate:201: base_axis_static_12mm:2 ↔ 3030_200:7
- Flush:65: 13to6_bearing:1 ↔ wormgear_axis_6mm:1
- Mate:202: 17HE19-2004S:1 ↔ wormgear_axis_6mm:1
- Mate:203: 3030_200:1 ↔ basis-bearing-3030-m6-holder:1
- Mate:204: 3030_260:3
- Mate:205 (6 mm): ax4_holder_asm:1 ↔ ax4:1
